# Autodesk Inventor assembly: Foot_front_frame_WearingImage
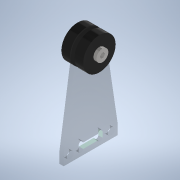
[picture p0: Inventor's stored thumbnail of the model, 180x180]
Saved by Autodesk Inventor 2022 (Build 260153000, 153)
## iProperties
Created: 2022-03-16
Part Number: Foot_front_frame_WearingImage
Document SubType Name: Assembly
Designer: Masato Kubotera
Author: Masato Kubotera
## Documents named in this file (5)
- C:\Users\Masato\Documents\Inventor\CIT Brains_Inventor\SUSTAINA-OP\OptionParts\SandBlastingJig\Foot_front_frame_WearingImage.iam
- C:\Users\Masato\Documents\Inventor\CIT Brains_Inventor\SUSTAINA-OP\LowerBody\Foot\Foot_front_frame.ipt
- C:\Users\Masato\Documents\Inventor\CIT Brains_Inventor\SUSTAINA-OP\OptionParts\SandBlastingJig\Foot_front_frame_SandBlastingJig_back.ipt
- C:\Users\Masato\Documents\Inventor\CIT Brains_Inventor\SUSTAINA-OP\OptionParts\SandBlastingJig\Foot_front_frame_SandBlastingJig_front.ipt
- C:\Users\Masato\Documents\Inventor\CIT Brains_Inventor\SUSTAINA-OP\ReadyMade\Screw\M3-10.ipt
## Components (4 placed, 4 different names)
1. Foot_front_frame:1 — 挿入:1, 挿入:2
2. Foot_front_frame_SandBlastingJig_back:1 — 挿入:1, 挿入:3
3. Foot_front_frame_SandBlastingJig_front:1 — 挿入:2
4. M3-10:1 — 挿入:3
## Relationships (3: Insert 3)
- 挿入:1 [Insert]: Foot_front_frame:1 ↔ Foot_front_frame_SandBlastingJig_back:1
- 挿入:2 [Insert]: Foot_front_frame:1 ↔ Foot_front_frame_SandBlastingJig_front:1
- 挿入:3 [Insert]: Foot_front_frame_SandBlastingJig_back:1 ↔ M3-10:1
